# Autodesk Inventor assembly: Assembly1
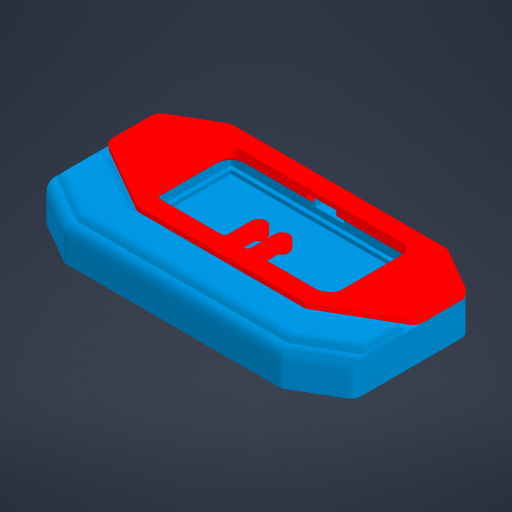
[picture p0: Inventor's stored thumbnail of the model, 512x512]
Saved by Autodesk Inventor 2023.4 (Build 274418000, 418)
## iProperties
Created: 2024-04-17
Part Number: Assembly1
Document SubType Name: Assembly
Designer: xSibe
Author: xSibe
## Documents named in this file (3)
- C:\.Laptop\.Work\Projects\Project Protocube\1 Autodesk\1 Cubes\Joystick\Joystick Enclosure.iam
- C:\.Laptop\.Work\Projects\Project Protocube\1 Autodesk\1 Cubes\Joystick\Joystick Bottom.ipt
- C:\.Laptop\.Work\Projects\Project Protocube\1 Autodesk\1 Cubes\Joystick\Joystick Top.ipt
## Components (2 placed, 2 different names)
1. Joystick Bottom:1 — Flush:1
2. Joystick Top:1 — Flush:1
## Relationships (1: Flush 1)
- Flush:1: Joystick Bottom:1 ↔ Joystick Top:1
